# Autodesk Inventor assembly: servocheck
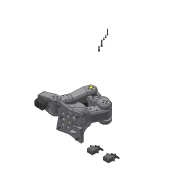
[picture p0: Inventor's stored thumbnail of the model, 180x180]
Saved by Autodesk Inventor 2018 (Build 220112000, 112)
## iProperties
Created: 2018-02-01
Part Number: servocheck
Document SubType Name: Assembly
Designer: Clevo
Author: Clevo
## Documents named in this file (22)
- E:\RobotArm\servocheck.iam
- E:\RobotArm\LX-16A.iam
- E:\RobotArm\base.ipt
- E:\RobotArm\52407bearing.ipt
- E:\RobotArm\table.ipt
- E:\RobotArm\arm2.ipt
- E:\RobotArm\arm2bearing_carrier.ipt
- E:\RobotArm\armbearing1.ipt
- E:\RobotArm\arm3.ipt
- E:\RobotArm\arm4.ipt
- E:\RobotArm\c_axisrot.ipt
- E:\RobotArm\bottomarm.iam
- E:\RobotArm\basebtm.ipt
- E:\RobotArm\arm6vers2.ipt
- E:\RobotArm\MG90servo_assembly.iam
- E:\RobotArm\91274A141_COATED ALLOY STEEL SOCKET HEAD CAP SCREW.ipt
- E:\RobotArm\91292A027_TYPE 18-8 SS SOCKET HEAD CAP SCREW.ipt
- E:\RobotArm\91292A123_TYPE 18-8 SS SOCKET HEAD CAP SCREW.ipt
- E:\RobotArm\91292A831_TYPE 18-8 SS SOCKET HEAD CAP SCREW.ipt
- E:\RobotArm\91292A832_TYPE 18-8 SS SOCKET HEAD CAP SCREW.ipt
- E:\RobotArm\92290A747_TYPE 316 SS SOCKET HEAD CAP SCREW.ipt
- E:\RobotArm\base_filler.ipt
## Components (47 placed, 21 different names)
1. LX-16A:1 [sub-assembly] — Mate:3, Mate:4, Angle:1, Mate:8
2. base:1 — Mate:3, Mate:4, Angle:1, Mate:5, Mate:6, Mate:52, Mate:53, Mate:54, Mate:82, Mate:83, Mate:84, Mate:85, Mate:86, Mate:87, Mate:88, Mate:89, Flush:5, Mate:107
3. 52407bearing:1 — Mate:5, Mate:6, Mate:7, Mate:106
4. table:1 — Mate:7, Mate:8, Mate:46, Mate:47, Mate:48
5. LX-16A:3 [sub-assembly] — Mate:18, Mate:19, Mate:41, Angle:11, Mate:51
6. arm2:1 — Mate:18, Mate:19, Mate:20, Mate:21, Mate:22, Mate:31, Mate:32, Angle:11, Mate:51
7. arm2bearing_carrier:1 — Mate:20, Mate:21, Mate:22, Mate:23, Mate:24, Angle:12
8. armbearing1:1 — Mate:23, Mate:24, Mate:38
9. LX-16A:4 [sub-assembly] — Mate:35, Mate:36, Angle:8
10. arm4:1 — Mate:28, Mate:29, Angle:6, Mate:31, Mate:32, Mate:49, Mate:50, Mate:98, Mate:99, Mate:100, Mate:101, Mate:102, Mate:103, Mate:104, Mate:105
11. LX-16A:5 [sub-assembly] — Mate:28, Mate:29, Angle:6
12. LX-16A:6 [sub-assembly] — Mate:55, Mate:56, Angle:13
13. arm3:1 — Mate:35, Mate:36, Angle:8, Mate:44, Mate:45, Flush:4, Angle:12, Mate:57, Mate:58
14. c_axisrot:1 — Mate:38, Mate:41, Mate:44, Mate:45, Flush:4
15. bottomarm:1 [sub-assembly] — Mate:46, Mate:47, Mate:48, Mate:49, Mate:50, Angle:10, Mate:59, Mate:60, Mate:61, Mate:62, Mate:64, Mate:67, Mate:68, Mate:69, Mate:70, Mate:71, Mate:72, Mate:73, Mate:74, Mate:75, Mate:76, Mate:77, Mate:78, Mate:79, Mate:80, Mate:81, Mate:90, Mate:91, Mate:92, Mate:93, Mate:94, Mate:95, Mate:96, Mate:97
16. basebtm:1 — Mate:52, Mate:53, Mate:54
17. arm6vers2:1 — Mate:55, Mate:56, Angle:13, Mate:57, Mate:58
18. MG90servo_assembly:1 [sub-assembly]
19. MG90servo_assembly:2 [sub-assembly]
20. 91274A141_COATED ALLOY STEEL SOCKET HEAD CAP SCREW:1 — Mate:82, Mate:88
21. 91292A027_TYPE 18-8 SS SOCKET HEAD CAP SCREW:1
22. 91292A123_TYPE 18-8 SS SOCKET HEAD CAP SCREW:1
23. 91292A831_TYPE 18-8 SS SOCKET HEAD CAP SCREW:1
24. 91292A832_TYPE 18-8 SS SOCKET HEAD CAP SCREW:1
25. 92290A747_TYPE 316 SS SOCKET HEAD CAP SCREW:1
26. 91292A831_TYPE 18-8 SS SOCKET HEAD CAP SCREW:2 — Mate:59, Mate:68
27. 91292A831_TYPE 18-8 SS SOCKET HEAD CAP SCREW:3 — Mate:62, Mate:70
28. 91292A831_TYPE 18-8 SS SOCKET HEAD CAP SCREW:4 — Mate:61, Mate:69
29. 91292A831_TYPE 18-8 SS SOCKET HEAD CAP SCREW:5 — Mate:60, Mate:67
30. 91292A831_TYPE 18-8 SS SOCKET HEAD CAP SCREW:9 — Mate:64, Mate:77
31. 91292A831_TYPE 18-8 SS SOCKET HEAD CAP SCREW:10 — Mate:71, Mate:76
32. 91292A831_TYPE 18-8 SS SOCKET HEAD CAP SCREW:11 — Mate:72, Mate:75
33. 91292A831_TYPE 18-8 SS SOCKET HEAD CAP SCREW:12 — Mate:73, Mate:74
34. 91292A123_TYPE 18-8 SS SOCKET HEAD CAP SCREW:2 — Mate:78, Mate:79
35. 91292A123_TYPE 18-8 SS SOCKET HEAD CAP SCREW:3 — Mate:80, Mate:81
36. 91274A141_COATED ALLOY STEEL SOCKET HEAD CAP SCREW:2 — Mate:83, Mate:89
37. 91274A141_COATED ALLOY STEEL SOCKET HEAD CAP SCREW:3 — Mate:85, Mate:86
38. 91274A141_COATED ALLOY STEEL SOCKET HEAD CAP SCREW:4 — Mate:84, Mate:87
39. 91292A027_TYPE 18-8 SS SOCKET HEAD CAP SCREW:2 — Mate:90, Mate:94
40. 91292A027_TYPE 18-8 SS SOCKET HEAD CAP SCREW:3 — Mate:91, Mate:96
41. 91292A027_TYPE 18-8 SS SOCKET HEAD CAP SCREW:4 — Mate:93, Mate:95
42. 91292A027_TYPE 18-8 SS SOCKET HEAD CAP SCREW:5 — Mate:92, Mate:97
43. 91292A027_TYPE 18-8 SS SOCKET HEAD CAP SCREW:6 — Mate:98, Mate:102
44. 91292A027_TYPE 18-8 SS SOCKET HEAD CAP SCREW:7 — Mate:101, Mate:103
45. 91292A027_TYPE 18-8 SS SOCKET HEAD CAP SCREW:8 — Mate:99, Mate:105
46. 91292A027_TYPE 18-8 SS SOCKET HEAD CAP SCREW:9 — Mate:100, Mate:104
47. base_filler:1 — Flush:5, Mate:106, Mate:107
## Relationships (91: Mate 82, Angle 7, Flush 2)
- Mate:3: LX-16A:1 ↔ base:1
- Mate:4: LX-16A:1 ↔ base:1
- Angle:1 (270 deg): LX-16A:1 ↔ base:1
- Mate:5: base:1 ↔ 52407bearing:1
- Mate:6: base:1 ↔ 52407bearing:1
- Mate:7: 52407bearing:1 ↔ table:1
- Mate:8: LX-16A:1 ↔ table:1
- Mate:18: LX-16A:3 ↔ arm2:1
- Mate:19: LX-16A:3 ↔ arm2:1
- Mate:20: arm2:1 ↔ arm2bearing_carrier:1
- Mate:21: arm2:1 ↔ arm2bearing_carrier:1
- Mate:22: arm2:1 ↔ arm2bearing_carrier:1
- Mate:23: arm2bearing_carrier:1 ↔ armbearing1:1
- Mate:24: arm2bearing_carrier:1 ↔ armbearing1:1
- Mate:28: arm4:1 ↔ LX-16A:5
- Mate:29: arm4:1 ↔ LX-16A:5
- Angle:6 (90 deg): arm4:1 ↔ LX-16A:5
- Mate:31: arm2:1 ↔ arm4:1
- Mate:32 (0.25 mm): arm2:1 ↔ arm4:1
- Mate:35: LX-16A:4 ↔ arm3:1
- Mate:36: LX-16A:4 ↔ arm3:1
- Angle:8 (0 deg): LX-16A:4 ↔ arm3:1
- Mate:38: armbearing1:1 ↔ c_axisrot:1
- Mate:41: LX-16A:3 ↔ c_axisrot:1
- Mate:44 (0.05 mm): arm3:1 ↔ c_axisrot:1
- Mate:45 (0.05 mm): arm3:1 ↔ c_axisrot:1
- Flush:4: arm3:1 ↔ c_axisrot:1
- Mate:46: table:1 ↔ bottomarm:1
- Mate:47: table:1 ↔ bottomarm:1
- Mate:48: table:1 ↔ bottomarm:1
- Mate:49: arm4:1 ↔ bottomarm:1
- Mate:50: arm4:1 ↔ bottomarm:1
- Angle:10 (0 deg): bottomarm:1
- Angle:11 (270 deg): LX-16A:3 ↔ arm2:1
- Mate:51 (0.0883 mm): LX-16A:3 ↔ arm2:1
- Mate:52: base:1 ↔ basebtm:1
- Mate:53: base:1 ↔ basebtm:1
- Mate:54: base:1 ↔ basebtm:1
- Angle:12 (0 deg): arm2bearing_carrier:1 ↔ arm3:1
- Mate:55: LX-16A:6 ↔ arm6vers2:1
- Mate:56: LX-16A:6 ↔ arm6vers2:1
- Angle:13 (-90 deg): LX-16A:6 ↔ arm6vers2:1
- Mate:57: arm3:1 ↔ arm6vers2:1
- Mate:58 (0.25 mm): arm3:1 ↔ arm6vers2:1
- Mate:59: bottomarm:1 ↔ 91292A831_TYPE 18-8 SS SOCKET HEAD CAP SCREW:2
- Mate:60: bottomarm:1 ↔ 91292A831_TYPE 18-8 SS SOCKET HEAD CAP SCREW:5
- Mate:61: bottomarm:1 ↔ 91292A831_TYPE 18-8 SS SOCKET HEAD CAP SCREW:4
- Mate:62: bottomarm:1 ↔ 91292A831_TYPE 18-8 SS SOCKET HEAD CAP SCREW:3
- Mate:64: bottomarm:1 ↔ 91292A831_TYPE 18-8 SS SOCKET HEAD CAP SCREW:9
- Mate:67: bottomarm:1 ↔ 91292A831_TYPE 18-8 SS SOCKET HEAD CAP SCREW:5
- Mate:68: bottomarm:1 ↔ 91292A831_TYPE 18-8 SS SOCKET HEAD CAP SCREW:2
- Mate:69: bottomarm:1 ↔ 91292A831_TYPE 18-8 SS SOCKET HEAD CAP SCREW:4
- Mate:70: bottomarm:1 ↔ 91292A831_TYPE 18-8 SS SOCKET HEAD CAP SCREW:3
- Mate:71: bottomarm:1 ↔ 91292A831_TYPE 18-8 SS SOCKET HEAD CAP SCREW:10
- Mate:72: bottomarm:1 ↔ 91292A831_TYPE 18-8 SS SOCKET HEAD CAP SCREW:11
- Mate:73: bottomarm:1 ↔ 91292A831_TYPE 18-8 SS SOCKET HEAD CAP SCREW:12
- Mate:74: bottomarm:1 ↔ 91292A831_TYPE 18-8 SS SOCKET HEAD CAP SCREW:12
- Mate:75: bottomarm:1 ↔ 91292A831_TYPE 18-8 SS SOCKET HEAD CAP SCREW:11
- Mate:76: bottomarm:1 ↔ 91292A831_TYPE 18-8 SS SOCKET HEAD CAP SCREW:10
- Mate:77: bottomarm:1 ↔ 91292A831_TYPE 18-8 SS SOCKET HEAD CAP SCREW:9
- Mate:78: bottomarm:1 ↔ 91292A123_TYPE 18-8 SS SOCKET HEAD CAP SCREW:2
- Mate:79: bottomarm:1 ↔ 91292A123_TYPE 18-8 SS SOCKET HEAD CAP SCREW:2
- Mate:80: bottomarm:1 ↔ 91292A123_TYPE 18-8 SS SOCKET HEAD CAP SCREW:3
- Mate:81: bottomarm:1 ↔ 91292A123_TYPE 18-8 SS SOCKET HEAD CAP SCREW:3
- Mate:82: base:1 ↔ 91274A141_COATED ALLOY STEEL SOCKET HEAD CAP SCREW:1
- Mate:83: base:1 ↔ 91274A141_COATED ALLOY STEEL SOCKET HEAD CAP SCREW:2
- Mate:84: base:1 ↔ 91274A141_COATED ALLOY STEEL SOCKET HEAD CAP SCREW:4
- Mate:85: base:1 ↔ 91274A141_COATED ALLOY STEEL SOCKET HEAD CAP SCREW:3
- Mate:86: base:1 ↔ 91274A141_COATED ALLOY STEEL SOCKET HEAD CAP SCREW:3
- Mate:87: base:1 ↔ 91274A141_COATED ALLOY STEEL SOCKET HEAD CAP SCREW:4
- Mate:88: base:1 ↔ 91274A141_COATED ALLOY STEEL SOCKET HEAD CAP SCREW:1
- Mate:89: base:1 ↔ 91274A141_COATED ALLOY STEEL SOCKET HEAD CAP SCREW:2
- Mate:90: bottomarm:1 ↔ 91292A027_TYPE 18-8 SS SOCKET HEAD CAP SCREW:2
- Mate:91: bottomarm:1 ↔ 91292A027_TYPE 18-8 SS SOCKET HEAD CAP SCREW:3
- Mate:92: bottomarm:1 ↔ 91292A027_TYPE 18-8 SS SOCKET HEAD CAP SCREW:5
- Mate:93: bottomarm:1 ↔ 91292A027_TYPE 18-8 SS SOCKET HEAD CAP SCREW:4
- Mate:94: bottomarm:1 ↔ 91292A027_TYPE 18-8 SS SOCKET HEAD CAP SCREW:2
- Mate:95: bottomarm:1 ↔ 91292A027_TYPE 18-8 SS SOCKET HEAD CAP SCREW:4
- Mate:96: bottomarm:1 ↔ 91292A027_TYPE 18-8 SS SOCKET HEAD CAP SCREW:3
- Mate:97: bottomarm:1 ↔ 91292A027_TYPE 18-8 SS SOCKET HEAD CAP SCREW:5
- Mate:98: arm4:1 ↔ 91292A027_TYPE 18-8 SS SOCKET HEAD CAP SCREW:6
- Mate:99: arm4:1 ↔ 91292A027_TYPE 18-8 SS SOCKET HEAD CAP SCREW:8
- Mate:100: arm4:1 ↔ 91292A027_TYPE 18-8 SS SOCKET HEAD CAP SCREW:9
- Mate:101: arm4:1 ↔ 91292A027_TYPE 18-8 SS SOCKET HEAD CAP SCREW:7
- Mate:102: arm4:1 ↔ 91292A027_TYPE 18-8 SS SOCKET HEAD CAP SCREW:6
- Mate:103: arm4:1 ↔ 91292A027_TYPE 18-8 SS SOCKET HEAD CAP SCREW:7
- Mate:104: arm4:1 ↔ 91292A027_TYPE 18-8 SS SOCKET HEAD CAP SCREW:9
- Mate:105: arm4:1 ↔ 91292A027_TYPE 18-8 SS SOCKET HEAD CAP SCREW:8
- Flush:5: base:1 ↔ base_filler:1
- Mate:106: 52407bearing:1 ↔ base_filler:1
- Mate:107: base:1 ↔ base_filler:1
